# Autodesk Inventor assembly: Assembly5
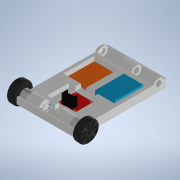
[picture p0: Inventor's stored thumbnail of the model, 180x180]
Saved by Autodesk Inventor 2022 (Build 260153000, 153)
## iProperties
Created: 2022-02-11
Part Number: Assembly5
Document SubType Name: Assembly
Designer: matys
Author: matys
## Documents named in this file (7)
- C:\Users\matys\Desktop\Práce4tak\Inventor\Assembly5.iam
- C:\Users\matys\Desktop\Práce4tak\Inventor\zakladna3.ipt
- C:\Users\matys\Desktop\Práce4tak\Inventor\motor.ipt
- C:\Users\matys\Desktop\Práce4tak\Inventor\L298N.ipt
- C:\Users\matys\Desktop\Práce4tak\Inventor\baterka.ipt
- C:\Users\matys\Desktop\Práce4tak\Inventor\podložka na arduino.ipt
- C:\Users\matys\Desktop\Práce4tak\Inventor\kolo.ipt
## Components (8 placed, 6 different names)
1. zakladna3:1 — Mate:3, Mate:5, Mate:6, Mate:7, Mate:8, Mate:9, Mate:10, Mate:11, Mate:12, Mate:13, Mate:14, Mate:15, Mate:16
2. motor:1 — Mate:15, Mate:16, Mate:17, Mate:18
3. motor:2 — Mate:3, Mate:14, Mate:19, Mate:20
4. L298N:1 — Mate:5, Mate:6, Mate:7
5. baterka:1 — Mate:8, Mate:9, Mate:10
6. podložka na arduino:1 — Mate:11, Mate:12, Mate:13
7. kolo:1 — Mate:19, Mate:20
8. kolo:2 — Mate:17, Mate:18
## Relationships (17: Mate 17)
- Mate:3: zakladna3:1 ↔ motor:2
- Mate:5: zakladna3:1 ↔ L298N:1
- Mate:6: zakladna3:1 ↔ L298N:1
- Mate:7: zakladna3:1 ↔ L298N:1
- Mate:8: zakladna3:1 ↔ baterka:1
- Mate:9: zakladna3:1 ↔ baterka:1
- Mate:10: zakladna3:1 ↔ baterka:1
- Mate:11: zakladna3:1 ↔ podložka na arduino:1
- Mate:12: zakladna3:1 ↔ podložka na arduino:1
- Mate:13: zakladna3:1 ↔ podložka na arduino:1
- Mate:14: zakladna3:1 ↔ motor:2
- Mate:15: zakladna3:1 ↔ motor:1
- Mate:16: zakladna3:1 ↔ motor:1
- Mate:17: motor:1 ↔ kolo:2
- Mate:18: motor:1 ↔ kolo:2
- Mate:19: motor:2 ↔ kolo:1
- Mate:20: motor:2 ↔ kolo:1
